# Autodesk Inventor assembly: robotface
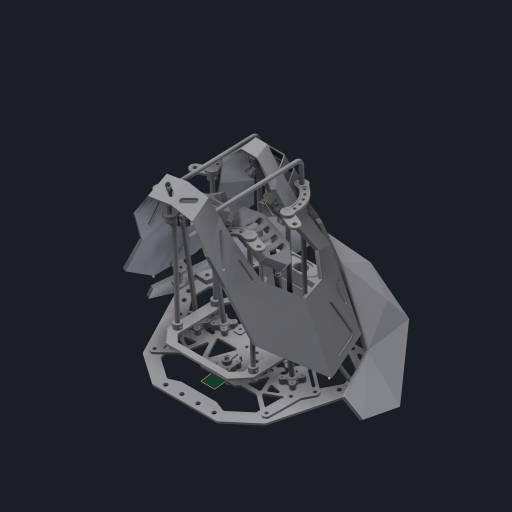
[picture p0: Inventor's stored thumbnail of the model, 512x512]
Saved by Autodesk Inventor 2023 (Build 270158000, 158)
## iProperties
Created: 2021-06-30
Part Number: robotface
Document SubType Name: Assembly
Designer: valer
Author: valer
## Documents named in this file (36)
- C:\Users\valer\Desktop\str1ker\cad\head\Head.iam
- C:\Users\valer\Desktop\str1ker\cad\head\Head.ipt
- C:\Users\valer\Desktop\str1ker\cad\external\HingedThreadedStandoffPart2.ipt
- C:\Users\valer\Desktop\str1ker\cad\external\HingedThreadedStandoffPart1.ipt
- C:\Users\valer\Desktop\str1ker\cad\head\TongueMount.ipt
- C:\Users\valer\Desktop\str1ker\cad\head\HeadMount.ipt
- C:\Users\valer\Desktop\str1ker\cad\external\LinearBearing-1612-0612-0035.ipt
- C:\Users\valer\Desktop\str1ker\cad\external\ClampingHub1301-0016-0012.ipt
- C:\Users\valer\Desktop\str1ker\cad\external\UJoint6D\UJoint6D-Body-4003-1006-1006.ipt
- C:\Users\valer\Desktop\str1ker\cad\external\UJoint6D\UJoint6D-CenterDrive-4003-1006-1006.ipt
- C:\Users\valer\Desktop\str1ker\cad\external\UJoint6D\UJoint6D-Screw.ipt
- C:\Users\valer\Desktop\str1ker\cad\external\SetScrewLiteHub-1308-0016-0006.ipt
- C:\Users\valer\Desktop\str1ker\cad\external\ShaftD6-Short-2101-0006-0020.ipt
- C:\Users\valer\Desktop\str1ker\cad\external\SetScrewHub-1300-0016-1006.ipt
- C:\Users\valer\Desktop\str1ker\cad\external\ShaftD6Female-632Female.ipt
- C:\Users\valer\Desktop\str1ker\cad\external\ShaftD6-2101-0006-0160.ipt
- C:\Users\valer\Desktop\str1ker\cad\head\HeadTongueMount.ipt
- C:\Users\valer\Desktop\str1ker\cad\external\Rod4mm.ipt
- C:\Users\valer\Desktop\str1ker\cad\head\NoseBentBar.ipt
- C:\Users\valer\Desktop\str1ker\cad\head\HeadTopConnector.ipt
- C:\Users\valer\Desktop\str1ker\cad\external\UJointSq-4005-0016-0001\4005-0016-0001 Outer Shell.ipt
- C:\Users\valer\Desktop\str1ker\cad\external\RodEndFixed-2434K495_CORROSION-RESISTANT FULLY THREADED ROD END BOLT.ipt
- C:\Users\valer\Desktop\str1ker\cad\external\StandoffM4-1501-0006-0420.ipt
- C:\Users\valer\Desktop\str1ker\cad\head\NoseInsideConnector.ipt
- C:\Users\valer\Desktop\str1ker\cad\external\Part2^3mm U-Joint.ipt
- C:\Users\valer\Desktop\str1ker\cad\external\Part1^3mm U-Joint.ipt
- C:\Users\valer\Desktop\str1ker\cad\head\NoseCover.ipt
- C:\Users\valer\Desktop\str1ker\cad\head\NoseCoverSmall.ipt
- C:\Users\valer\Desktop\str1ker\cad\external\ShaftClamp6-6058N14.ipt
- C:\Users\valer\Desktop\str1ker\cad\head\MuzzleHeadMount.ipt
- C:\Users\valer\Desktop\str1ker\cad\external\ShaftD6-2100-0006-0200.ipt
- C:\Users\valer\Desktop\str1ker\cad\head\MuzzleHeadConnector.ipt
- C:\Users\valer\Desktop\str1ker\cad\VacuumTubeHolder.iam
- C:\Users\valer\Desktop\str1ker\cad\FaceTubeConnector.ipt
- C:\Users\valer\Desktop\str1ker\cad\head\HeadJaw.ipt
- C:\Users\valer\Desktop\str1ker\cad\external\DepthSensor\PrimeSenseCarmine1.09.ipt
## Components (107 placed, 35 different names)
1. Head:1 — Mate:7, Mate:8, Mate:9, Mate:10, Mate:11, Mate:12, Angle:3, Mate:18, Mate:19, Mate:20, Mate:25, Mate:26, Mate:90, Mate:91, Mate:92, Mate:93, Angle:18, Angle:20, Mate:132, Mate:133, Angle:28, Mate:189, Mate:190, Angle:35, Angle:36, Mate:205, Angle:41, Mate:242, Mate:244, Mate:245, Mate:246, Mate:247, Mate:254, Mate:255, Angle:47, Mate:278, Mate:282, Mate:368, Mate:369, Angle:58, Mate:380, Mate:381, Mate:382, Mate:383, Mate:386, Mate:387, Mate:389, Mate:404, Mate:405, Mate:414, Mate:415, Mate:416, Mate:417, Mate:418, Mate:419, Mate:463, Mate:465, Mate:469, Mate:474, Mate:509, Mate:512, Mate:517
2. HingedThreadedStandoffPart2:1 — Mate:1, Mate:2, Flush:1, Angle:4, Mate:284
3. HingedThreadedStandoffPart1:1 — Mate:1, Mate:2, Mate:7, Mate:8
4. HingedThreadedStandoffPart2:2 — Mate:3, Mate:4, Mate:9, Mate:10
5. HingedThreadedStandoffPart1:2 — Mate:3, Mate:4, Flush:1
6. HingedThreadedStandoffPart2:3 — Mate:5, Mate:6, Mate:11, Mate:12, Angle:3, Mate:60, Mate:61
7. HingedThreadedStandoffPart1:3 — Mate:5, Mate:6, Angle:4
8. HingedThreadedStandoffPart2:4 — Mate:18, Mate:19, Mate:20, Mate:21, Mate:22
9. HingedThreadedStandoffPart1:4 — Mate:21, Mate:22, Mate:89
10. HingedThreadedStandoffPart2:5 — Mate:25, Mate:26
11. HingedThreadedStandoffPart1:5 — Mate:85, Mate:86
12. TongueMount:2 — Mate:278, Mate:281, Mate:283, Mate:284, Flush:24
13. HeadMount:1 — Mate:110, Mate:111, Mate:112, Flush:12, Mate:210, Mate:211, Mate:214, Mate:215
14. LinearBearing-1612-0612-0035:1 — Mate:300, Flush:25
15. ClampingHub1301-0016-0012:1 — Mate:115, Mate:282, Mate:300, Flush:25
16. SetScrewLiteHub-1308-0016-0006:1 — Mate:65, Mate:67, Mate:281, Angle:53, Flush:24
17. HingedThreadedStandoffPart2:6 — Mate:60, Mate:61, Mate:283
18. ShaftD6-Short-2101-0006-0020:1 — Mate:65, Mate:67, Angle:51, Mate:297, Flush:22
19. ShaftD6-2101-0006-0160:2 — Mate:87, Angle:16
20. ShaftD6-2101-0006-0160:3
21. SetScrewHub-1300-0016-1006:1
22. SetScrewHub-1300-0016-1006:2
23. ShaftD6Female-632Female:1 — Mate:85, Mate:86
24. ShaftD6Female-632Female:2 — Mate:87, Mate:89, Angle:16
25. HingedThreadedStandoffPart2:9 — Mate:92, Mate:93, Mate:96, Mate:97
26. HingedThreadedStandoffPart2:10 — Mate:90, Mate:91, Mate:94, Mate:95
27. HingedThreadedStandoffPart2:11 — Mate:94, Mate:95, Mate:98, Mate:99
28. HingedThreadedStandoffPart2:12 — Mate:96, Mate:97, Mate:100, Mate:101
29. ShaftD6Female-632Female:3 — Mate:98, Mate:99, Mate:102, Angle:17, Mate:103, Angle:18
30. ShaftD6Female-632Female:4 — Mate:100, Mate:101, Mate:104, Angle:19, Angle:20, Mate:105
31. ShaftD6-2101-0006-0160:4 — Mate:102, Angle:17, Mate:103, Mate:106, Angle:21
32. ShaftD6-2101-0006-0160:5 — Mate:104, Angle:19, Mate:105, Mate:107, Angle:22
33. SetScrewHub-1300-0016-1006:3 — Mate:106, Angle:21, Mate:116
34. SetScrewHub-1300-0016-1006:4 — Mate:107, Angle:22
35. HeadTongueMount:1 — Mate:110, Mate:111, Mate:112, Mate:115, Mate:116, Mate:204, Mate:483
36. Rod4mm:1 — Mate:132
37. Rod4mm:2 — Mate:133
38. SetScrewLiteHub-1308-0016-0006:2 — Mate:151, Flush:5, Mate:153, Angle:26, Mate:242, Mate:370, Mate:371
39. UJoint6D-Body-4003-1006-1006:5 — Angle:28
40. UJoint6D-CenterDrive-4003-1006-1006:3
41. UJoint6D-Screw:11
42. UJoint6D-Body-4003-1006-1006:6 — Mate:152, Angle:25, Mate:153, Angle:26
43. UJoint6D-Screw:12
44. UJoint6D-Screw:13
45. UJoint6D-Screw:14
46. ShaftD6-Short-2101-0006-0020:2 — Mate:151, Flush:5, Mate:152, Angle:25
47. NoseBentBar:1 — Mate:189, Angle:36, Flush:13, Flush:14
48. NoseBentBar:2 — Mate:190, Angle:35, Flush:13
49. HeadTopConnector:1 — Flush:12, Flush:14
50. 4005-0016-0001 Outer Shell:1 — Mate:204, Mate:205
51. RodEndFixed-2434K495_CORROSION-RESISTANT FULLY THREADED ROD END BOLT:1 — Mate:210, Mate:211, Angle:41, Angle:42
52. RodEndFixed-2434K495_CORROSION-RESISTANT FULLY THREADED ROD END BOLT:3 — Mate:214, Mate:215, Angle:42
53. StandoffM4-1501-0006-0420:1 — Mate:244, Mate:245
54. StandoffM4-1501-0006-0420:2 — Mate:246, Mate:247
55. HingedThreadedStandoffPart2:13 — Mate:256, Mate:257
56. HingedThreadedStandoffPart1:6 — Mate:254, Mate:255, Angle:47
57. ShaftD6Female-632Female:5 — Mate:256, Mate:257
58. UJoint6D-Body-4003-1006-1006:12 — Angle:51, Mate:297, Flush:22, Angle:53
59. UJoint6D-Screw:24
60. UJoint6D-Screw:26
61. NoseInsideConnector:1 — Mate:368, Mate:369, Angle:58, Mate:370, Mate:371
62. Part2^3mm U-Joint:1 — Mate:372, Mate:373, Mate:374, Mate:375
63. Part1^3mm U-Joint:1 — Mate:372, Mate:373
64. Part1^3mm U-Joint:2 — Mate:374, Mate:375, Mate:380, Mate:381
65. Part2^3mm U-Joint:2
66. Part1^3mm U-Joint:3
67. Part1^3mm U-Joint:4 — Mate:382, Mate:383
68. NoseCover:1 — Mate:386, Mate:387, Flush:29, Mate:388
69. NoseCoverSmall:1 — Flush:29, Mate:388, Mate:389
70. ShaftD6-2100-0006-0200:1 — Mate:432, Mate:436, Mate:482
71. ShaftClamp6-6058N14:1 — Mate:404, Mate:405
72. ShaftD6-2100-0006-0200:2 — Mate:441, Mate:443, Mate:458
73. ShaftClamp6-6058N14:2 — Mate:464
74. ShaftD6-2100-0006-0200:3 — Mate:445, Mate:447, Mate:466
75. ShaftClamp6-6058N14:3
76. ShaftClamp6-6058N14:4 — Mate:414, Mate:415
77. ShaftClamp6-6058N14:5 — Mate:416, Mate:417
78. ShaftD6-2100-0006-0200:4 — Mate:437, Mate:439, Mate:480
79. ShaftClamp6-6058N14:6 — Mate:418, Mate:419
80. ShaftD6-2100-0006-0200:5 — Mate:449, Mate:451, Mate:475
81. ShaftClamp6-6058N14:7 — Mate:476
82. ShaftD6-2100-0006-0200:6 — Mate:453, Mate:455, Mate:470
83. ShaftClamp6-6058N14:8 — Mate:471
84. MuzzleHeadMount:1 — Mate:428, Mate:429, Mate:480, Mate:481, Mate:482, Mate:484, Mate:485, Mate:486, Mate:487, Mate:488, Mate:489, Mate:490, Mate:491, Mate:492, Mate:493, Mate:494, Mate:495
85. MuzzleHeadConnector:1 — Mate:428, Mate:429, Mate:481, Mate:483
86. ShaftClamp6-6058N14:9 — Mate:432, Mate:485
87. ShaftClamp6-6058N14:10 — Mate:436, Mate:486
88. ShaftClamp6-6058N14:12 — Mate:437, Mate:487
89. ShaftClamp6-6058N14:13 — Mate:439, Mate:484
90. ShaftClamp6-6058N14:14 — Mate:441, Mate:492
91. ShaftClamp6-6058N14:15 — Mate:443, Mate:493
92. ShaftClamp6-6058N14:16 — Mate:445, Mate:494
93. ShaftClamp6-6058N14:17 — Mate:447, Mate:488
94. ShaftClamp6-6058N14:18 — Mate:449, Mate:495
95. ShaftClamp6-6058N14:19 — Mate:451, Mate:491
96. ShaftClamp6-6058N14:20 — Mate:453, Mate:490
97. ShaftClamp6-6058N14:21 — Mate:455, Mate:489
98. VacuumTubeHolder:1 [sub-assembly] — Mate:467, Mate:468
99. VacuumTubeHolder:2 [sub-assembly] — Mate:461, Mate:462
100. VacuumTubeHolder:3 [sub-assembly] — Mate:477, Mate:478
101. VacuumTubeHolder:4 [sub-assembly] — Mate:472, Mate:473
102. BackSideConnector:1 — Mate:458, Mate:461, Mate:462, Mate:463, Mate:464
103. BackSideConnector:2 — Mate:465, Mate:466, Mate:467, Mate:468
104. BackSideConnector:3 — Mate:469, Mate:470, Mate:471, Mate:472, Mate:473
105. BackSideConnector:4 — Mate:474, Mate:475, Mate:476, Mate:477, Mate:478
106. HeadJaw:1 — Mate:510, Mate:515, Mate:517
107. PrimeSenseCarmine1.09:1 — Angle:59
## Relationships (243: Mate 202, Angle 28, Flush 13)
- Mate:1: HingedThreadedStandoffPart2:1 ↔ HingedThreadedStandoffPart1:1
- Mate:2: HingedThreadedStandoffPart2:1 ↔ HingedThreadedStandoffPart1:1
- Mate:3: HingedThreadedStandoffPart2:2 ↔ HingedThreadedStandoffPart1:2
- Mate:4: HingedThreadedStandoffPart2:2 ↔ HingedThreadedStandoffPart1:2
- Mate:5: HingedThreadedStandoffPart2:3 ↔ HingedThreadedStandoffPart1:3
- Mate:6: HingedThreadedStandoffPart2:3 ↔ HingedThreadedStandoffPart1:3
- Mate:7: Head:1 ↔ HingedThreadedStandoffPart1:1
- Mate:8: Head:1 ↔ HingedThreadedStandoffPart1:1
- Mate:9: Head:1 ↔ HingedThreadedStandoffPart2:2
- Mate:10: Head:1 ↔ HingedThreadedStandoffPart2:2
- Mate:11: Head:1 ↔ HingedThreadedStandoffPart2:3
- Mate:12: Head:1 ↔ HingedThreadedStandoffPart2:3
- Angle:3 (0 deg): Head:1 ↔ HingedThreadedStandoffPart2:3
- Mate:18: Head:1 ↔ HingedThreadedStandoffPart2:4
- Mate:19: Head:1 ↔ HingedThreadedStandoffPart2:4
- Mate:20: Head:1 ↔ HingedThreadedStandoffPart2:4
- Mate:21: HingedThreadedStandoffPart2:4 ↔ HingedThreadedStandoffPart1:4
- Mate:22: HingedThreadedStandoffPart2:4 ↔ HingedThreadedStandoffPart1:4
- [Mate]: HingedThreadedStandoffPart2:5 ↔ HingedThreadedStandoffPart1:5
- [Mate]: HingedThreadedStandoffPart2:5 ↔ HingedThreadedStandoffPart1:5
- Mate:25: Head:1 ↔ HingedThreadedStandoffPart2:5
- Mate:26: Head:1 ↔ HingedThreadedStandoffPart2:5
- Flush:1: HingedThreadedStandoffPart2:1 ↔ HingedThreadedStandoffPart1:2
- Angle:4 (0 deg): HingedThreadedStandoffPart2:1 ↔ HingedThreadedStandoffPart1:3
- Mate:60: HingedThreadedStandoffPart2:3 ↔ HingedThreadedStandoffPart2:6
- Mate:61: HingedThreadedStandoffPart2:3 ↔ HingedThreadedStandoffPart2:6
- Mate:65: SetScrewLiteHub-1308-0016-0006:1 ↔ ShaftD6-Short-2101-0006-0020:1
- Mate:67 (-7 mm): SetScrewLiteHub-1308-0016-0006:1 ↔ ShaftD6-Short-2101-0006-0020:1
- [Mate]: HingedThreadedStandoffPart1:4 ↔ ShaftD6-2101-0006-0160:2
- [Angle] (0 deg): HeadMount:1 ↔ ShaftD6-2101-0006-0160:2
- [Mate]: HingedThreadedStandoffPart1:5 ↔ ShaftD6-2101-0006-0160:3
- [Angle] (0 deg): HeadMount:1 ↔ ShaftD6-2101-0006-0160:3
- [Mate]: ShaftD6-2101-0006-0160:2 ↔ SetScrewHub-1300-0016-1006:1
- [Mate]: ShaftD6-2101-0006-0160:3 ↔ SetScrewHub-1300-0016-1006:2
- [Angle] (0 deg): ShaftD6-2101-0006-0160:2 ↔ SetScrewHub-1300-0016-1006:1
- [Angle] (0 deg): ShaftD6-2101-0006-0160:3 ↔ SetScrewHub-1300-0016-1006:2
- [Angle] (0 deg): Head:1 ↔ ShaftD6-2101-0006-0160:2
- [Angle] (0 deg): Head:1 ↔ ShaftD6-2101-0006-0160:3
- [Mate]: ShaftD6-2101-0006-0160:3 ↔ ShaftD6Female-632Female:1
- [Angle] (0 deg): ShaftD6-2101-0006-0160:3 ↔ ShaftD6Female-632Female:1
- [Mate]: ShaftD6-2101-0006-0160:3 ↔ ShaftD6Female-632Female:1
- Mate:85: HingedThreadedStandoffPart1:5 ↔ ShaftD6Female-632Female:1
- Mate:86: HingedThreadedStandoffPart1:5 ↔ ShaftD6Female-632Female:1
- Mate:87: ShaftD6-2101-0006-0160:2 ↔ ShaftD6Female-632Female:2
- Mate:89: HingedThreadedStandoffPart1:4 ↔ ShaftD6Female-632Female:2
- Angle:16 (0 deg): ShaftD6-2101-0006-0160:2 ↔ ShaftD6Female-632Female:2
- Mate:90: Head:1 ↔ HingedThreadedStandoffPart2:10
- Mate:91: Head:1 ↔ HingedThreadedStandoffPart2:10
- Mate:92: Head:1 ↔ HingedThreadedStandoffPart2:9
- Mate:93: Head:1 ↔ HingedThreadedStandoffPart2:9
- Mate:94: HingedThreadedStandoffPart2:10 ↔ HingedThreadedStandoffPart2:11
- Mate:95: HingedThreadedStandoffPart2:10 ↔ HingedThreadedStandoffPart2:11
- Mate:96: HingedThreadedStandoffPart2:9 ↔ HingedThreadedStandoffPart2:12
- Mate:97: HingedThreadedStandoffPart2:9 ↔ HingedThreadedStandoffPart2:12
- Mate:98: HingedThreadedStandoffPart2:11 ↔ ShaftD6Female-632Female:3
- Mate:99: HingedThreadedStandoffPart2:11 ↔ ShaftD6Female-632Female:3
- Mate:100: HingedThreadedStandoffPart2:12 ↔ ShaftD6Female-632Female:4
- Mate:101: HingedThreadedStandoffPart2:12 ↔ ShaftD6Female-632Female:4
- Mate:102: ShaftD6Female-632Female:3 ↔ ShaftD6-2101-0006-0160:4
- Angle:17 (0 deg): ShaftD6Female-632Female:3 ↔ ShaftD6-2101-0006-0160:4
- Mate:103: ShaftD6Female-632Female:3 ↔ ShaftD6-2101-0006-0160:4
- Angle:18 (180 deg): Head:1 ↔ ShaftD6Female-632Female:3
- Mate:104: ShaftD6Female-632Female:4 ↔ ShaftD6-2101-0006-0160:5
- Angle:19 (0 deg): ShaftD6Female-632Female:4 ↔ ShaftD6-2101-0006-0160:5
- Angle:20 (180 deg): Head:1 ↔ ShaftD6Female-632Female:4
- Mate:105: ShaftD6Female-632Female:4 ↔ ShaftD6-2101-0006-0160:5
- Mate:106: ShaftD6-2101-0006-0160:4 ↔ SetScrewHub-1300-0016-1006:3
- Angle:21 (180 deg): ShaftD6-2101-0006-0160:4 ↔ SetScrewHub-1300-0016-1006:3
- Mate:107: ShaftD6-2101-0006-0160:5 ↔ SetScrewHub-1300-0016-1006:4
- Angle:22 (180 deg): ShaftD6-2101-0006-0160:5 ↔ SetScrewHub-1300-0016-1006:4
- Mate:110: HeadMount:1 ↔ HeadTongueMount:1
- Mate:111: HeadMount:1 ↔ HeadTongueMount:1
- Mate:112: HeadMount:1 ↔ HeadTongueMount:1
- Mate:115: ClampingHub1301-0016-0012:1 ↔ HeadTongueMount:1
- Mate:116: SetScrewHub-1300-0016-1006:3 ↔ HeadTongueMount:1
- Mate:132: Head:1 ↔ Rod4mm:1
- Mate:133: Head:1 ↔ Rod4mm:2
- [Mate]: UJoint6D-CenterDrive-4003-1006-1006:3 ↔ UJoint6D-Body-4003-1006-1006:6
- [Mate]: UJoint6D-CenterDrive-4003-1006-1006:3 ↔ UJoint6D-Body-4003-1006-1006:6
- [Mate]: UJoint6D-Body-4003-1006-1006:5 ↔ UJoint6D-CenterDrive-4003-1006-1006:3
- [Mate]: UJoint6D-Body-4003-1006-1006:5 ↔ UJoint6D-CenterDrive-4003-1006-1006:3
- [Mate]: UJoint6D-Body-4003-1006-1006:5 ↔ UJoint6D-Screw:11
- [Mate]: UJoint6D-Body-4003-1006-1006:5 ↔ UJoint6D-Screw:11
- [Mate]: UJoint6D-Body-4003-1006-1006:5 ↔ UJoint6D-Screw:13
- [Mate]: UJoint6D-Body-4003-1006-1006:5 ↔ UJoint6D-Screw:13
- [Mate]: UJoint6D-Body-4003-1006-1006:6 ↔ UJoint6D-Screw:12
- [Mate]: UJoint6D-Body-4003-1006-1006:6 ↔ UJoint6D-Screw:12
- [Mate]: UJoint6D-Body-4003-1006-1006:6 ↔ UJoint6D-Screw:14
- [Mate]: UJoint6D-Body-4003-1006-1006:6 ↔ UJoint6D-Screw:14
- Mate:151: SetScrewLiteHub-1308-0016-0006:2 ↔ ShaftD6-Short-2101-0006-0020:2
- Flush:5: SetScrewLiteHub-1308-0016-0006:2 ↔ ShaftD6-Short-2101-0006-0020:2
- Mate:152: UJoint6D-Body-4003-1006-1006:6 ↔ ShaftD6-Short-2101-0006-0020:2
- Angle:25 (180 deg): UJoint6D-Body-4003-1006-1006:6 ↔ ShaftD6-Short-2101-0006-0020:2
- Mate:153: SetScrewLiteHub-1308-0016-0006:2 ↔ UJoint6D-Body-4003-1006-1006:6
- Angle:26 (0 deg): SetScrewLiteHub-1308-0016-0006:2 ↔ UJoint6D-Body-4003-1006-1006:6
- Angle:28 (0 deg): Head:1 ↔ UJoint6D-Body-4003-1006-1006:5
- Mate:189: Head:1 ↔ NoseBentBar:1
- Mate:190: Head:1 ↔ NoseBentBar:2
- Flush:12: HeadMount:1 ↔ HeadTopConnector:1
- Angle:35 (0 deg): Head:1 ↔ NoseBentBar:2
- Angle:36 (0 deg): Head:1 ↔ NoseBentBar:1
- Flush:13: NoseBentBar:1 ↔ NoseBentBar:2
- Flush:14: NoseBentBar:1 ↔ HeadTopConnector:1
- Mate:204: HeadTongueMount:1 ↔ 4005-0016-0001 Outer Shell:1
- Mate:205: Head:1 ↔ 4005-0016-0001 Outer Shell:1
- Mate:210: HeadMount:1 ↔ RodEndFixed-2434K495_CORROSION-RESISTANT FULLY THREADED ROD END BOLT:1
- Mate:211 (-17.78 mm): HeadMount:1 ↔ RodEndFixed-2434K495_CORROSION-RESISTANT FULLY THREADED ROD END BOLT:1
- Angle:41 (0 deg): Head:1 ↔ RodEndFixed-2434K495_CORROSION-RESISTANT FULLY THREADED ROD END BOLT:1
- Mate:214: HeadMount:1 ↔ RodEndFixed-2434K495_CORROSION-RESISTANT FULLY THREADED ROD END BOLT:3
- Mate:215 (-17.78 mm): HeadMount:1 ↔ RodEndFixed-2434K495_CORROSION-RESISTANT FULLY THREADED ROD END BOLT:3
- Angle:42 (0 deg): RodEndFixed-2434K495_CORROSION-RESISTANT FULLY THREADED ROD END BOLT:1 ↔ RodEndFixed-2434K495_CORROSION-RESISTANT FULLY THREADED ROD END BOLT:3
- Mate:242: Head:1 ↔ SetScrewLiteHub-1308-0016-0006:2
- Mate:244: Head:1 ↔ StandoffM4-1501-0006-0420:1
- Mate:245: Head:1 ↔ StandoffM4-1501-0006-0420:1
- Mate:246: Head:1 ↔ StandoffM4-1501-0006-0420:2
- Mate:247: Head:1 ↔ StandoffM4-1501-0006-0420:2
- [Mate]: HingedThreadedStandoffPart2:13 ↔ HingedThreadedStandoffPart1:6
- [Mate]: HingedThreadedStandoffPart2:13 ↔ HingedThreadedStandoffPart1:6
- Mate:254: Head:1 ↔ HingedThreadedStandoffPart1:6
- Mate:255: Head:1 ↔ HingedThreadedStandoffPart1:6
- Angle:47 (0 deg): Head:1 ↔ HingedThreadedStandoffPart1:6
- Mate:256: HingedThreadedStandoffPart2:13 ↔ ShaftD6Female-632Female:5
- Mate:257: HingedThreadedStandoffPart2:13 ↔ ShaftD6Female-632Female:5
- Mate:278: Head:1 ↔ TongueMount:2
- Mate:281: TongueMount:2 ↔ SetScrewLiteHub-1308-0016-0006:1
- Mate:282: Head:1 ↔ ClampingHub1301-0016-0012:1
- Mate:283: TongueMount:2 ↔ HingedThreadedStandoffPart2:6
- Mate:284: HingedThreadedStandoffPart2:1 ↔ TongueMount:2
- [Mate]: UJoint6D-Body-4003-1006-1006:12 ↔ UJoint6D-Screw:24
- [Mate]: UJoint6D-Body-4003-1006-1006:12 ↔ UJoint6D-Screw:24
- [Mate]: UJoint6D-Body-4003-1006-1006:12 ↔ UJoint6D-Screw:26
- [Mate]: UJoint6D-Body-4003-1006-1006:12 ↔ UJoint6D-Screw:26
- Angle:51 (0 deg): ShaftD6-Short-2101-0006-0020:1 ↔ UJoint6D-Body-4003-1006-1006:12
- Mate:297: ShaftD6-Short-2101-0006-0020:1 ↔ UJoint6D-Body-4003-1006-1006:12
- Flush:22: ShaftD6-Short-2101-0006-0020:1 ↔ UJoint6D-Body-4003-1006-1006:12
- Angle:53 (0 deg): SetScrewLiteHub-1308-0016-0006:1 ↔ UJoint6D-Body-4003-1006-1006:12
- Mate:300: LinearBearing-1612-0612-0035:1 ↔ ClampingHub1301-0016-0012:1
- Flush:24: TongueMount:2 ↔ SetScrewLiteHub-1308-0016-0006:1
- Flush:25 (6 mm): LinearBearing-1612-0612-0035:1 ↔ ClampingHub1301-0016-0012:1
- Mate:368: Head:1 ↔ NoseInsideConnector:1
- Mate:369: Head:1 ↔ NoseInsideConnector:1
- Angle:58 (0 deg): Head:1 ↔ NoseInsideConnector:1
- Mate:370: SetScrewLiteHub-1308-0016-0006:2 ↔ NoseInsideConnector:1
- Mate:371: SetScrewLiteHub-1308-0016-0006:2 ↔ NoseInsideConnector:1
- Mate:372: Part2^3mm U-Joint:1 ↔ Part1^3mm U-Joint:1
- Mate:373 (0.15 mm): Part2^3mm U-Joint:1 ↔ Part1^3mm U-Joint:1
- Mate:374: Part2^3mm U-Joint:1 ↔ Part1^3mm U-Joint:2
- Mate:375 (0.15 mm): Part2^3mm U-Joint:1 ↔ Part1^3mm U-Joint:2
- [Mate]: Part2^3mm U-Joint:2 ↔ Part1^3mm U-Joint:3
- [Mate] (0.15 mm): Part2^3mm U-Joint:2 ↔ Part1^3mm U-Joint:3
- [Mate]: Part2^3mm U-Joint:2 ↔ Part1^3mm U-Joint:4
- [Mate] (0.15 mm): Part2^3mm U-Joint:2 ↔ Part1^3mm U-Joint:4
- Mate:380: Head:1 ↔ Part1^3mm U-Joint:2
- Mate:381: Head:1 ↔ Part1^3mm U-Joint:2
- Mate:382: Head:1 ↔ Part1^3mm U-Joint:4
- Mate:383: Head:1 ↔ Part1^3mm U-Joint:4
- Mate:386: Head:1 ↔ NoseCover:1
- Mate:387: Head:1 ↔ NoseCover:1
- Flush:29: NoseCover:1 ↔ NoseCoverSmall:1
- Mate:388 (10 mm): NoseCover:1 ↔ NoseCoverSmall:1
- Mate:389: Head:1 ↔ NoseCoverSmall:1
- Mate:404: Head:1 ↔ ShaftClamp6-6058N14:1
- Mate:405: Head:1 ↔ ShaftClamp6-6058N14:1
- [Mate]: Head:1 ↔ ShaftD6-2100-0006-0200:1
- [Mate]: Head:1 ↔ ShaftD6-2100-0006-0200:1
- [Mate]: Head:1 ↔ ShaftD6-2100-0006-0200:2
- [Mate]: ShaftD6-2100-0006-0200:2 ↔ ShaftClamp6-6058N14:2
- [Flush]: Head:1 ↔ ShaftD6-2100-0006-0200:2
- [Mate]: ShaftD6-2100-0006-0200:3 ↔ ShaftClamp6-6058N14:3
- [Mate]: Head:1 ↔ ShaftD6-2100-0006-0200:3
- [Flush]: Head:1 ↔ ShaftD6-2100-0006-0200:3
- Mate:414: Head:1 ↔ ShaftClamp6-6058N14:4
- Mate:415: Head:1 ↔ ShaftClamp6-6058N14:4
- Mate:416: Head:1 ↔ ShaftClamp6-6058N14:5
- Mate:417: Head:1 ↔ ShaftClamp6-6058N14:5
- Mate:418: Head:1 ↔ ShaftClamp6-6058N14:6
- Mate:419: Head:1 ↔ ShaftClamp6-6058N14:6
- [Mate]: ShaftD6-2100-0006-0200:4 ↔ ShaftClamp6-6058N14:6
- [Mate]: Head:1 ↔ ShaftD6-2100-0006-0200:4
- [Mate]: ShaftD6-2100-0006-0200:5 ↔ ShaftClamp6-6058N14:7
- [Mate]: Head:1 ↔ ShaftD6-2100-0006-0200:5
- [Flush]: Head:1 ↔ ShaftD6-2100-0006-0200:5
- [Mate]: ShaftD6-2100-0006-0200:6 ↔ ShaftClamp6-6058N14:8
- [Mate]: Head:1 ↔ ShaftD6-2100-0006-0200:6
- [Flush]: Head:1 ↔ ShaftD6-2100-0006-0200:6
- Mate:428: MuzzleHeadMount:1 ↔ MuzzleHeadConnector:1
- Mate:429: MuzzleHeadMount:1 ↔ MuzzleHeadConnector:1
- Mate:432: ShaftD6-2100-0006-0200:1 ↔ ShaftClamp6-6058N14:9
- Mate:436: ShaftD6-2100-0006-0200:1 ↔ ShaftClamp6-6058N14:10
- Mate:437: ShaftD6-2100-0006-0200:4 ↔ ShaftClamp6-6058N14:12
- Mate:439: ShaftD6-2100-0006-0200:4 ↔ ShaftClamp6-6058N14:13
- Mate:441: ShaftD6-2100-0006-0200:2 ↔ ShaftClamp6-6058N14:14
- Mate:443: ShaftD6-2100-0006-0200:2 ↔ ShaftClamp6-6058N14:15
- Mate:445: ShaftD6-2100-0006-0200:3 ↔ ShaftClamp6-6058N14:16
- Mate:447: ShaftD6-2100-0006-0200:3 ↔ ShaftClamp6-6058N14:17
- Mate:449: ShaftD6-2100-0006-0200:5 ↔ ShaftClamp6-6058N14:18
- Mate:451: ShaftD6-2100-0006-0200:5 ↔ ShaftClamp6-6058N14:19
- Mate:453: ShaftD6-2100-0006-0200:6 ↔ ShaftClamp6-6058N14:20
- Mate:455: ShaftD6-2100-0006-0200:6 ↔ ShaftClamp6-6058N14:21
- Mate:458: ShaftD6-2100-0006-0200:2 ↔ BackSideConnector:1
- Mate:461: VacuumTubeHolder:2 ↔ BackSideConnector:1
- Mate:462: VacuumTubeHolder:2 ↔ BackSideConnector:1
- Mate:463: Head:1 ↔ BackSideConnector:1
- Mate:464: ShaftClamp6-6058N14:2 ↔ BackSideConnector:1
- Mate:465: Head:1 ↔ BackSideConnector:2
- Mate:466: ShaftD6-2100-0006-0200:3 ↔ BackSideConnector:2
- Mate:467: VacuumTubeHolder:1 ↔ BackSideConnector:2
- Mate:468: VacuumTubeHolder:1 ↔ BackSideConnector:2
- Mate:469: Head:1 ↔ BackSideConnector:3
- Mate:470: ShaftD6-2100-0006-0200:6 ↔ BackSideConnector:3
- Mate:471: ShaftClamp6-6058N14:8 ↔ BackSideConnector:3
- Mate:472: VacuumTubeHolder:4 ↔ BackSideConnector:3
- Mate:473: VacuumTubeHolder:4 ↔ BackSideConnector:3
- Mate:474: Head:1 ↔ BackSideConnector:4
- Mate:475: ShaftD6-2100-0006-0200:5 ↔ BackSideConnector:4
- Mate:476: ShaftClamp6-6058N14:7 ↔ BackSideConnector:4
- Mate:477: VacuumTubeHolder:3 ↔ BackSideConnector:4
- Mate:478: VacuumTubeHolder:3 ↔ BackSideConnector:4
- Mate:480: ShaftD6-2100-0006-0200:4 ↔ MuzzleHeadMount:1
- Mate:481: MuzzleHeadMount:1 ↔ MuzzleHeadConnector:1
- Mate:482: ShaftD6-2100-0006-0200:1 ↔ MuzzleHeadMount:1
- Mate:483: HeadTongueMount:1 ↔ MuzzleHeadConnector:1
- Mate:484: MuzzleHeadMount:1 ↔ ShaftClamp6-6058N14:13
- Mate:485: MuzzleHeadMount:1 ↔ ShaftClamp6-6058N14:9
- Mate:486: MuzzleHeadMount:1 ↔ ShaftClamp6-6058N14:10
- Mate:487: MuzzleHeadMount:1 ↔ ShaftClamp6-6058N14:12
- Mate:488: MuzzleHeadMount:1 ↔ ShaftClamp6-6058N14:17
- Mate:489: MuzzleHeadMount:1 ↔ ShaftClamp6-6058N14:21
- Mate:490: MuzzleHeadMount:1 ↔ ShaftClamp6-6058N14:20
- Mate:491: MuzzleHeadMount:1 ↔ ShaftClamp6-6058N14:19
- Mate:492: MuzzleHeadMount:1 ↔ ShaftClamp6-6058N14:14
- Mate:493: MuzzleHeadMount:1 ↔ ShaftClamp6-6058N14:15
- Mate:494: MuzzleHeadMount:1 ↔ ShaftClamp6-6058N14:16
- Mate:495: MuzzleHeadMount:1 ↔ ShaftClamp6-6058N14:18
- Mate:509: Head:1
- Mate:510: HeadJaw:1
- Mate:511
- Mate:512: Head:1
- Mate:514
- Mate:515: HeadJaw:1
- Mate:516
- Mate:517: Head:1 ↔ HeadJaw:1
- Angle:59 (180 deg): PrimeSenseCarmine1.09:1
## Named parameters: d60_d58 = 0 mm, d61_d59 = 0 mm, d275_d245_d146 = 0 mm, d276_d246_d147 = 0 mm, d277_d247_d148 = 0 mm, d278_d248_d149 = 0 mm, d279_d249_d150 = 0 mm, d280_d250_d151 = 0 mm, d281_d251_d152 = 0 mm, d282_d252_d153 = 0 mm, d283_d253_d154 = 0 mm, d284_d254_d155 = 0 mm, d285_d255_d156 = 0 mm, d286_d256_d157 = 0 mm, d466_d58 = 0 mm, d467_d59 = 0 mm, d520_d253_d154 = 0 mm, d521_d254_d155 = 0 mm, d522_d255_d156 = 0 mm, d523_d256_d157 = 0 mm, d629_d625 = 0 mm, d630_d626 = 0.15 mm, d631_d627 = 0 mm, d632_d628 = 0.15 mm, d678_d675 = 0 mm, d692_d678_d675 = 0 mm, d696_d692_d678_d675 = 0 mm
